# Autodesk Inventor assembly: CAMERA ASSEMBLY
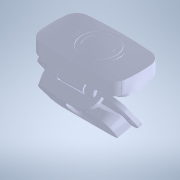
[picture p0: Inventor's stored thumbnail of the model, 180x180]
Saved by Autodesk Inventor 2020 (Build 240168000, 168)
## iProperties
Created: 2014-06-29
Part Number: CAMERA ASSEMBLY
Description: STEP AP214
Document SubType Name: Assembly
Designer: haya
Sending System: SolidWorks 2013
Preprocessor: SwSTEP 2.0
Title: CAMERA ASSEMBLY.STEP
Revision Number: ANY
## Documents named in this file (6)
- C:\Users\haya\Desktop\IRC\camera\CAMERA ASSEMBLY.iam
- C:\Users\haya\Desktop\IRC\camera\camera-1B.ipt
- C:\Users\haya\Desktop\IRC\camera\camera-1A.ipt
- C:\Users\haya\Desktop\IRC\camera\camera-2.ipt
- C:\Users\haya\Desktop\IRC\camera\camera-3.ipt
- C:\Users\haya\Desktop\IRC\camera\camera-4.ipt
## Components (5 placed, 5 different names)
1. camera-1B_1 — 挿入:3
2. camera-1A_2 — 挿入:2, 挿入:3
3. camera-2_3 — 挿入:1, 挿入:2, 角度:1
4. camera-3_4 — 挿入:1, 角度:1
5. camera-4_5
## Relationships (4: Insert 3, Angle 1)
- 挿入:1 [Insert]: camera-2_3 ↔ camera-3_4
- 挿入:2 [Insert]: camera-1A_2 ↔ camera-2_3
- 角度:1 [Angle] (180 deg): camera-2_3 ↔ camera-3_4
- 挿入:3 [Insert]: camera-1B_1 ↔ camera-1A_2
